# Autodesk Inventor assembly: Assembly_Cube_v4_Beamsplittercube_30mm
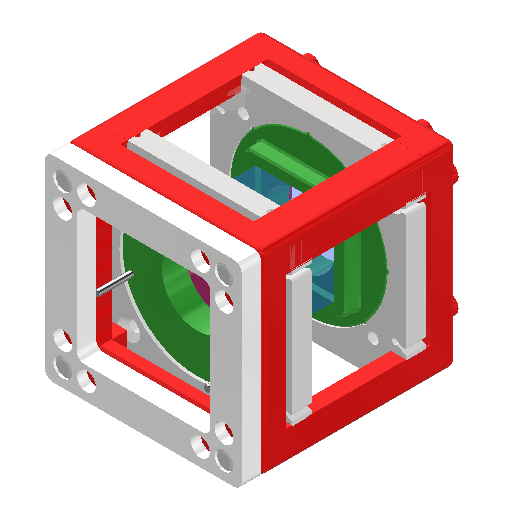
[picture p0: Inventor's stored thumbnail of the model, 512x512]
Saved by Autodesk Inventor 2025.1 (Build 291241000, 241)
## iProperties
Created: 2024-10-03
Part Number: Assembly_Cube_v4_Beamsplittercube_30mm
Document SubType Name: Assembly
Designer: diederichbenedict
Author: diederichbenedict
## Documents named in this file (5)
- C:\Users\Muriel\Documents\GitHub\TechnicalDocs-openUC2-QBox\Production_Files\CAD_Files\INVENTOR\Assembly_Cube_v4_Beamsplittercube_30mm.iam
- C:\Users\Muriel\Documents\GitHub\TechnicalDocs-openUC2-QBox\Production_Files\CAD_Files\INVENTOR\Assembly_Cube_v4.iam
- C:\Users\Muriel\Documents\GitHub\TechnicalDocs-openUC2-QBox\Production_Files\CAD_Files\INVENTOR\00_Beamsplitter_20mm.ipt
- C:\Users\Muriel\Documents\GitHub\TechnicalDocs-openUC2-QBox\Production_Files\CAD_Files\INVENTOR\10_Insert_v4.ipt
- C:\Users\Muriel\Documents\GitHub\TechnicalDocs-openUC2-QBox\Production_Files\CAD_Files\INVENTOR\20_Cube_4_insert_beamsplitter_20mm.ipt
## Components (6 placed, 4 different names)
1. Assembly_Cube_v4:1 [sub-assembly] — Mate:1, Mate:2, Flush:1, Flush:2, Flush:3, Mate:3, Angle:1, Mate:4
2. 00_Beamsplitter_20mm:1 — Flush:1, Flush:2, Flush:3
3. 10_Insert_v4:1 — Mate:3, Angle:1, Mate:4, Flush:4, Flush:5
4. 20_Cube_4_insert_beamsplitter_20mm:1 — Flush:4, Flush:5
5. 10_Insert_v4:2
6. 20_Cube_4_insert_beamsplitter_20mm:2
## Component patterns: (2 elements, first: 10_Insert_v4:1 + 20_Cube_4_insert_beamsplitter_20mm:1)
## Relationships (10: Flush 5, Mate 4, Angle 1)
- Mate:1: Assembly_Cube_v4:1
- Mate:2: Assembly_Cube_v4:1
- Flush:1: Assembly_Cube_v4:1 ↔ 00_Beamsplitter_20mm:1
- Flush:2: Assembly_Cube_v4:1 ↔ 00_Beamsplitter_20mm:1
- Flush:3: Assembly_Cube_v4:1 ↔ 00_Beamsplitter_20mm:1
- Mate:3: Assembly_Cube_v4:1 ↔ 10_Insert_v4:1
- Angle:1 (360 deg): Assembly_Cube_v4:1 ↔ 10_Insert_v4:1
- Mate:4: Assembly_Cube_v4:1 ↔ 10_Insert_v4:1
- Flush:4: 10_Insert_v4:1 ↔ 20_Cube_4_insert_beamsplitter_20mm:1
- Flush:5: 10_Insert_v4:1 ↔ 20_Cube_4_insert_beamsplitter_20mm:1
